# Autodesk Inventor assembly: Assy_curve_module
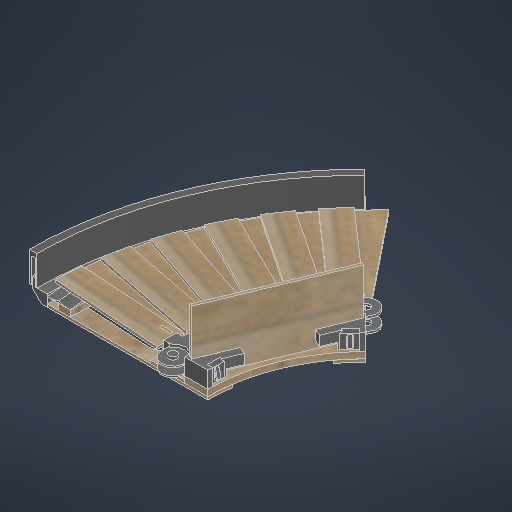
[picture p0: Inventor's stored thumbnail of the model, 512x512]
Saved by Autodesk Inventor 2027.1 (Build 311270010, 270A)
## iProperties
Created: 2025-09-28
Part Number: Assy_curve_module
Document SubType Name: Assembly
Designer: hibik
Author: hibik
## Documents named in this file (12)
- C:\Users\takuya\Documents\D2_conveyor\curve_module\Assy_curve_module.iam
- C:\Users\takuya\Documents\D2_conveyor\curve_module\base.ipt
- C:\Users\takuya\Documents\D2_conveyor\curve_module\back_under.ipt
- C:\Users\takuya\Documents\D2_conveyor\curve_module\back_upper.ipt
- C:\Users\takuya\Documents\D2_conveyor\curve_module\front.ipt
- C:\Users\takuya\Documents\D2_conveyor\curve_module\belt_rail.ipt
- C:\Users\takuya\Documents\D2_conveyor\belt\belt_curve.iam
- C:\Users\takuya\Documents\D2_conveyor\connectors\connector_male_bend_left.ipt
- C:\Users\takuya\Documents\D2_conveyor\connectors\connector_male_bend_right.ipt
- C:\Users\takuya\Documents\D2_conveyor\curve_module\wall.ipt
- C:\Users\takuya\Documents\D2_conveyor\curve_module\front_rail.ipt
- C:\Users\takuya\Documents\D2_conveyor\curve_module\Rail_Wall.ipt
## Components (12 placed, 11 different names)
1. base:1 — 挿入:3, 挿入:5, フラッシュ:2, 角度:8, 正接:3
2. front:1 — 挿入:3, 角度:3, メイト:10, メイト:11, メイト:12
3. back_under:1 — 挿入:5, 角度:5, 挿入:7, フラッシュ:1, 挿入:8, 挿入:9, 正接:2, メイト:1, メイト:2, メイト:3, メイト:4, メイト:5, メイト:6, メイト:9
4. back_upper:1 — 角度:6, 挿入:9
5. base:2 — 挿入:7, フラッシュ:1
6. belt_rail:1 — 挿入:8, フラッシュ:2, 正接:1
7. belt_curve:1 [sub-assembly] — 正接:1, 正接:2, 角度:8, 正接:3
8. connector_male_bend_left:1 — メイト:2, メイト:3, メイト:6
9. connector_male_bend_right:1 — メイト:1, メイト:4, メイト:5, メイト:7, メイト:8
10. wall:1 — メイト:7, メイト:8, メイト:9
11. front_rail:1 — メイト:10, メイト:11, メイト:12, メイト:13, 正接:4, フラッシュ:3
12. Rail_Wall:1 — メイト:13, 正接:4, フラッシュ:3
## Relationships (30: Mate 13, Insert 5, Angle 4, Tangent 4, Flush 3, Symmetry 1)
- 挿入:3 [Insert]: base:1 ↔ front:1
- 角度:3 [Angle] (0 deg): front:1
- 挿入:5 [Insert]: base:1 ↔ back_under:1
- 角度:5 [Angle] (0 deg): back_under:1
- 角度:6 [Angle] (0 deg): back_upper:1
- 挿入:7 [Insert]: back_under:1 ↔ base:2
- フラッシュ:1 [Flush]: back_under:1 ↔ base:2
- 挿入:8 [Insert]: back_under:1 ↔ belt_rail:1
- フラッシュ:2 [Flush]: base:1 ↔ belt_rail:1
- 挿入:9 [Insert]: back_under:1 ↔ back_upper:1
- 正接:1 [Tangent]: belt_rail:1 ↔ belt_curve:1
- 正接:2 [Tangent]: back_under:1 ↔ belt_curve:1
- 角度:8 [Angle] (3.75 deg): base:1 ↔ belt_curve:1
- 正接:3 [Tangent] (-3.5 mm): base:1 ↔ belt_curve:1
- メイト:1 [Mate]: back_under:1 ↔ connector_male_bend_right:1
- メイト:2 [Mate]: back_under:1 ↔ connector_male_bend_left:1
- メイト:3 [Mate]: back_under:1 ↔ connector_male_bend_left:1
- メイト:4 [Mate]: back_under:1 ↔ connector_male_bend_right:1
- メイト:5 [Mate]: back_under:1 ↔ connector_male_bend_right:1
- メイト:6 [Mate]: back_under:1 ↔ connector_male_bend_left:1
- メイト:7 [Mate]: connector_male_bend_right:1 ↔ wall:1
- メイト:8 [Mate]: connector_male_bend_right:1 ↔ wall:1
- メイト:9 [Mate]: back_under:1 ↔ wall:1
- 対称度:1 [Symmetry]
- メイト:10 [Mate]: front:1 ↔ front_rail:1
- メイト:11 [Mate]: front:1 ↔ front_rail:1
- メイト:12 [Mate]: front:1 ↔ front_rail:1
- メイト:13 [Mate]: front_rail:1 ↔ Rail_Wall:1
- 正接:4 [Tangent]: front_rail:1 ↔ Rail_Wall:1
- フラッシュ:3 [Flush]: front_rail:1 ↔ Rail_Wall:1
